# Autodesk Inventor assembly: дрон сборка
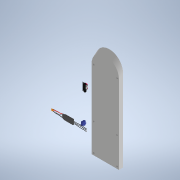
[picture p0: Inventor's stored thumbnail of the model, 180x180]
Saved by Autodesk Inventor 2022 (Build 260153000, 153)
## iProperties
Created: 2021-12-25
Part Number: дрон сборка
Document SubType Name: Assembly
Designer: Grigori
Author: Grigori
## Documents named in this file (17)
- C:\Users\User\Documents\GitHub\ModularDrone\Сборка\дрон сборка.iam
- C:\Users\User\Documents\GitHub\ModularDrone\Сборка\корпус.ipt
- C:\Users\User\Documents\GitHub\ModularDrone\PartsModels\Ardupilot\APM 2.5 Side Entry Case.ipt
- C:\Users\User\Documents\GitHub\ModularDrone\PartsModels\ESC\esc 80A.ipt
- C:\Users\User\Documents\GitHub\ModularDrone\PartsModels\GPS\PX4 Neo M8N GPS.ipt
- C:\Users\User\Documents\GitHub\ModularDrone\PartsModels\Servo\SG90\SG90 v1.ipt
- C:\Users\User\Documents\GitHub\ModularDrone\PartsModels\Telemetry\3D Robotics Radio Telemetry Kit.ipt
- C:\Users\User\Documents\GitHub\ModularDrone\PartsModels\Winch\Treuil Yeah racing\Treuil Yeah racing.ipt
- C:\Users\User\Documents\GitHub\ModularDrone\PartsModels\Box Battery\Сборка.ipt
- C:\Users\User\Documents\GitHub\ModularDrone\Сборка\Крышка на отсек с батареей.ipt
- C:\Users\Grigo\Documents\Inventor\Content Center Files\R2022\ru-RU\AS 1427(01)\AS 1427 - M3 x 10(3).ipt
- C:\Users\User\Documents\GitHub\ModularDrone\Сборка\Сборка крышка.iam
- C:\Users\User\Documents\Inventor\Content Center Files\R2022\ru-RU\DIN 976-1 A\DIN 976-1 - M5 x 60 - A.ipt
- C:\Users\User\Documents\GitHub\ModularDrone\Сборка\площадка.ipt
- C:\Users\User\Documents\GitHub\ModularDrone\Сборка\проставка.ipt
- C:\Users\User\Documents\GitHub\ModularDrone\PartsModels\power boars scheme v3 v2\power boars scheme v3.iam
- C:\Users\User\Documents\Inventor\Content Center Files\R2022\ru-RU\ANSI B 18.2.4.1 M(1)\ANSI B 18.2.4.1 M - M4 x 0,7Style 1.ipt
## Components (38 placed, 16 different names)
1. корпус:1 — Совмещение:1, Совмещение:2, Совмещение:3, С поворотом:1, С поворотом:2, Совмещение:4, Совмещение:5, Совмещение:6, Вставка:1, Вставка:2, Вставка:3, Вставка:4, Вставка:5
2. APM 2.5 Side Entry Case:1 — Жесткий:7
3. esc 80A:1
4. PX4 Neo M8N GPS:1 — Жесткий:9
5. SG90 v1:1
6. 3D Robotics Radio Telemetry Kit:1 — Жесткий:8
7. Treuil Yeah racing:1
8. Сборка:1 — Совмещение:1, Совмещение:2, Совмещение:3
9. Крышка на отсек с батареей:1 — С поворотом:1, С поворотом:2, С поворотом:3, С поворотом:4, Жесткий:2, С поворотом:5, Жесткий:3, Жесткий:4, Жесткий:5, Жесткий:6
10. AS 1427 - метрическая M3 x 10:1 — Жесткий:3
11. AS 1427 - метрическая M3 x 10:2 — Жесткий:2
12. AS 1427 - метрическая M3 x 10:3 — С поворотом:4
13. AS 1427 - метрическая M3 x 10:4 — Жесткий:5
14. AS 1427 - метрическая M3 x 10:5 — Жесткий:6
15. AS 1427 - метрическая M3 x 10:6 — С поворотом:5
16. AS 1427 - метрическая M3 x 10:7 — Жесткий:4
17. AS 1427 - метрическая M3 x 10:8 — С поворотом:3
18. Сборка крышка:1 [sub-assembly] — Совмещение:4, Совмещение:5, Совмещение:6
19. DIN 976-1 A M5 x 60:1 — Вставка:1, Вставка:7, Вставка:13
20. DIN 976-1 A M5 x 60:2 — Вставка:2, Вставка:6, Вставка:14
21. DIN 976-1 A M5 x 60:3 — Вставка:3, Вставка:8, Вставка:12
22. DIN 976-1 A M5 x 60:4 — Вставка:4, Вставка:9, Вставка:11
23. площадка:1 — Вставка:5, Жесткий:7
24. проставка:1 — Вставка:9
25. проставка:2 — Вставка:8
26. проставка:3 — Вставка:7, Вставка:10
27. проставка:4 — Вставка:6
28. площадка:2 — Вставка:10, Жесткий:8, Жесткий:9
29. проставка:5 — Вставка:12
30. проставка:6 — Вставка:13, Вставка:15
31. проставка:7 — Вставка:14
32. проставка:8 — Вставка:11
33. площадка:3 — Вставка:15, Жесткий:10, Вставка:16, Вставка:17, Вставка:18, Вставка:19
34. power boars scheme v3:1 [sub-assembly] — Жесткий:10
35. Шестигранная гайка метрическая M4 x 0,7:1 — Вставка:16
36. Шестигранная гайка метрическая M4 x 0,7:2 — Вставка:17
37. Шестигранная гайка метрическая M4 x 0,7:3 — Вставка:18
38. Шестигранная гайка метрическая M4 x 0,7:4 — Вставка:19
## Relationships (39: Insert 19, WeldJoint 9, Mate 6, RevoluteJoint 5)
- Совмещение:1 [Mate]: корпус:1 ↔ Сборка:1
- Совмещение:2 [Mate]: корпус:1 ↔ Сборка:1
- Совмещение:3 [Mate]: корпус:1 ↔ Сборка:1
- С поворотом:1 [RevoluteJoint]: корпус:1 ↔ Крышка на отсек с батареей:1
- С поворотом:2 [RevoluteJoint]: корпус:1 ↔ Крышка на отсек с батареей:1
- С поворотом:3 [RevoluteJoint]: Крышка на отсек с батареей:1 ↔ AS 1427 - метрическая M3 x 10:8
- С поворотом:4 [RevoluteJoint]: Крышка на отсек с батареей:1 ↔ AS 1427 - метрическая M3 x 10:3
- Жесткий:2 [WeldJoint]: Крышка на отсек с батареей:1 ↔ AS 1427 - метрическая M3 x 10:2
- С поворотом:5 [RevoluteJoint]: Крышка на отсек с батареей:1 ↔ AS 1427 - метрическая M3 x 10:6
- Жесткий:3 [WeldJoint]: Крышка на отсек с батареей:1 ↔ AS 1427 - метрическая M3 x 10:1
- Жесткий:4 [WeldJoint]: Крышка на отсек с батареей:1 ↔ AS 1427 - метрическая M3 x 10:7
- Жесткий:5 [WeldJoint]: Крышка на отсек с батареей:1 ↔ AS 1427 - метрическая M3 x 10:4
- Жесткий:6 [WeldJoint]: Крышка на отсек с батареей:1 ↔ AS 1427 - метрическая M3 x 10:5
- Совмещение:4 [Mate]: корпус:1 ↔ Сборка крышка:1
- Совмещение:5 [Mate]: корпус:1 ↔ Сборка крышка:1
- Совмещение:6 [Mate]: корпус:1 ↔ Сборка крышка:1
- Вставка:1 [Insert] (-46 mm): корпус:1 ↔ DIN 976-1 A M5 x 60:1
- Вставка:2 [Insert] (-46 mm): корпус:1 ↔ DIN 976-1 A M5 x 60:2
- Вставка:3 [Insert] (-46 mm): корпус:1 ↔ DIN 976-1 A M5 x 60:3
- Вставка:4 [Insert] (-46 mm): корпус:1 ↔ DIN 976-1 A M5 x 60:4
- Вставка:5 [Insert]: корпус:1 ↔ площадка:1
- Жесткий:7 [WeldJoint]: APM 2.5 Side Entry Case:1 ↔ площадка:1
- Вставка:6 [Insert] (15 mm): DIN 976-1 A M5 x 60:2 ↔ проставка:4
- Вставка:7 [Insert] (15 mm): DIN 976-1 A M5 x 60:1 ↔ проставка:3
- Вставка:8 [Insert] (15 mm): DIN 976-1 A M5 x 60:3 ↔ проставка:2
- Вставка:9 [Insert] (15 mm): DIN 976-1 A M5 x 60:4 ↔ проставка:1
- Вставка:10 [Insert]: проставка:3 ↔ площадка:2
- Жесткий:8 [WeldJoint]: 3D Robotics Radio Telemetry Kit:1 ↔ площадка:2
- Жесткий:9 [WeldJoint]: PX4 Neo M8N GPS:1 ↔ площадка:2
- Вставка:11 [Insert] (4 mm): DIN 976-1 A M5 x 60:4 ↔ проставка:8
- Вставка:12 [Insert] (4 mm): DIN 976-1 A M5 x 60:3 ↔ проставка:5
- Вставка:13 [Insert] (4 mm): DIN 976-1 A M5 x 60:1 ↔ проставка:6
- Вставка:14 [Insert] (4 mm): DIN 976-1 A M5 x 60:2 ↔ проставка:7
- Вставка:15 [Insert]: проставка:6 ↔ площадка:3
- Жесткий:10 [WeldJoint]: площадка:3 ↔ power boars scheme v3:1
- Вставка:16 [Insert]: площадка:3 ↔ Шестигранная гайка метрическая M4 x 0,7:1
- Вставка:17 [Insert]: площадка:3 ↔ Шестигранная гайка метрическая M4 x 0,7:2
- Вставка:18 [Insert]: площадка:3 ↔ Шестигранная гайка метрическая M4 x 0,7:3
- Вставка:19 [Insert]: площадка:3 ↔ Шестигранная гайка метрическая M4 x 0,7:4
